# Autodesk Inventor assembly: base mg996r 3mm frame middle
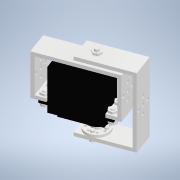
[picture p0: Inventor's stored thumbnail of the model, 180x180]
Saved by Autodesk Inventor 2021.4 (Build 254397000, 397)
## iProperties
Created: 2022-07-09
Part Number: base mg996r 3mm frame middle
Document SubType Name: Assembly
Designer: isamu
Author: isamu
## Documents named in this file (5)
- D:\personal_projects\robot\inventor\2021\base mg996r 3mm frame middle.iam
- D:\personal_projects\robot\inventor\2021\base mg996r 3mm frame with axis.iam
- D:\personal_projects\robot\exports\frames\servo frame mg996r.ipt
- D:\personal_projects\robot\exports\screws\m2 nuts.ipt
- D:\personal_projects\robot\exports\screws\m4 nuts.ipt
## Components (7 placed, 4 different names)
1. base mg996r 3mm frame with axis:1 [sub-assembly] — Mate:1, Mate:2, Mate:3
2. servo frame mg996r:1 — Insert:9, Insert:10, Insert:11, Insert:12, Insert:13, Mate:1, Mate:2, Mate:3
3. m2 nuts:1 — Insert:10
4. m2 nuts:2 — Insert:11
5. m2 nuts:3 — Insert:12
6. m2 nuts:4 — Insert:13
7. m4 nuts:1 — Insert:9
## Relationships (8: Insert 5, Mate 3)
- Insert:9: servo frame mg996r:1 ↔ m4 nuts:1
- Insert:10: servo frame mg996r:1 ↔ m2 nuts:1
- Insert:11: servo frame mg996r:1 ↔ m2 nuts:2
- Insert:12: servo frame mg996r:1 ↔ m2 nuts:3
- Insert:13: servo frame mg996r:1 ↔ m2 nuts:4
- Mate:1: base mg996r 3mm frame with axis:1 ↔ servo frame mg996r:1
- Mate:2: base mg996r 3mm frame with axis:1 ↔ servo frame mg996r:1
- Mate:3: base mg996r 3mm frame with axis:1 ↔ servo frame mg996r:1
